# Autodesk Inventor assembly: Acoplamiento
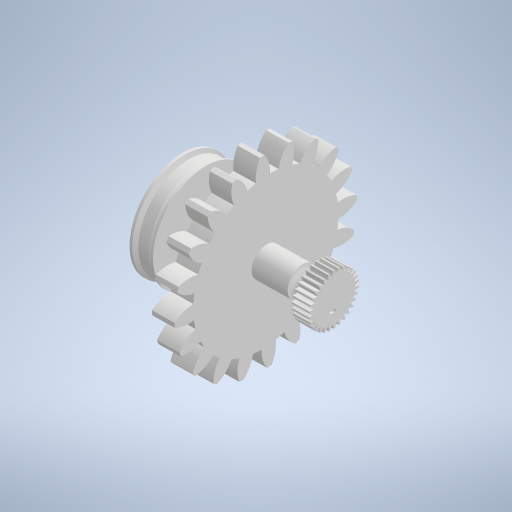
[picture p0: Inventor's stored thumbnail of the model, 512x512]
Saved by Autodesk Inventor 2024 (Build 280153000, 153)
## iProperties
Created: 2024-03-18
Part Number: Acoplamiento
Document SubType Name: Assembly
Designer: Eva Sinay
Author: Eva Sinay
## Documents named in this file (6)
- C:\Users\Eva Sinay\Documents\Acoplamiento.iam
- C:\Users\Eva Sinay\Desktop\CUÑA.ipt
- C:\Users\Eva Sinay\Desktop\EJE_CUÑEROS.ipt
- C:\Users\Eva Sinay\Desktop\POLEA.ipt
- C:\Users\Eva Sinay\Desktop\ENGRANE.ipt
- C:\Users\Eva Sinay\Desktop\Engrane Central.ipt
## Components (6 placed, 5 different names)
1. CUÑA:1 — Rígido:2, Tangente:1
2. CUÑA:2 — Rígido:1
3. EJE_CUÑEROS:1 — Rígido:1, Rígido:2, Tangente:1, De rotación:1, De rotación:2, De rotación:3
4. POLEA:1 — De rotación:1
5. ENGRANE:1 — De rotación:2
6. Engrane Central:1 — De rotación:3
## Relationships (6: RevoluteJoint 3, WeldJoint 2, Tangent 1)
- Rígido:1 [WeldJoint]: CUÑA:2 ↔ EJE_CUÑEROS:1
- Rígido:2 [WeldJoint]: CUÑA:1 ↔ EJE_CUÑEROS:1
- Tangente:1: CUÑA:1 ↔ EJE_CUÑEROS:1
- De rotación:1 [RevoluteJoint]: EJE_CUÑEROS:1 ↔ POLEA:1
- De rotación:2 [RevoluteJoint]: EJE_CUÑEROS:1 ↔ ENGRANE:1
- De rotación:3 [RevoluteJoint] (10 mm): EJE_CUÑEROS:1 ↔ Engrane Central:1
